# Autodesk Inventor assembly: Robot
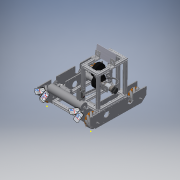
[picture p0: Inventor's stored thumbnail of the model, 180x180]
Saved by Autodesk Inventor 2017 (Build 210142000, 142)
## iProperties
Created: 2016-10-08
Part Number: Robot
Document SubType Name: Assembly
Designer: RoboticsUser
Author: RoboticsUser
## Documents named in this file (12)
- C:\Robotics\CAD\2016-17_CAD\Robot - CAD.iam
- C:\Robotics\CAD\COTSParts\Bosch Extrusion\Gusset 20x20 w screws.ipt
- C:\Robotics\CAD\COTSParts\Bosch Extrusion\Bosch 20x20 9 in - Copy.ipt
- C:\Robotics\CAD\COTSParts\Bosch Extrusion\Rexroth-6mmT-Nutm4.ipt
- C:\Robotics\CAD\COTSParts\Bosch Extrusion\Bosch 20x20 8.937in.ipt
- C:\Robotics\CAD\2016-17_CAD\ParticleLauncher2.0.iam
- C:\Robotics\CAD\2016-17_CAD\Deflecter.ipt
- C:\Robotics\CAD\COTSParts\Actobotics\585 parts\585424.ipt
- C:\Robotics\CAD\2016-17_CAD\WheelAssemble2.0.iam
- C:\Robotics\CAD\2016-17_CAD\RollerHolder.ipt
- C:\Robotics\CAD\2016-17_CAD\NewRoller.ipt
- C:\Robotics\CAD\COTSParts\Bosch Extrusion\Bosch 20x20 9 real.ipt
## Components (21 placed, 11 different names)
1. Bosch 20x20 9 in - Copy:1 — Mate:33, Flush:25, Flush:150, Mate:248, Flush:151, Flush:152, Mate:251, Flush:156, Flush:157, Mate:252, Flush:158
2. Rexroth-6mmT-Nutm4:1
3. Rexroth-6mmT-Nutm4:2 — Mate:33, Flush:25
4. Rexroth-6mmT-Nutm4:3
5. Bosch 20x20 9 in - Copy:2 — Mate:15, Flush:11, Mate:249, Flush:153, Flush:154, Mate:250, Flush:155, Flush:159
6. Rexroth-6mmT-Nutm4:4 — Insert:14
7. Rexroth-6mmT-Nutm4:5
8. Rexroth-6mmT-Nutm4:6 — Mate:15, Flush:11
9. Bosch 20x20 8.937in:4 — Mate:93, Flush:62, Flush:92, Flush:103, Flush:104, Mate:160
10. ParticleLauncher2.0:1 [sub-assembly] — Flush:103, Flush:104, Mate:160, Mate:174, Flush:113, Mate:245, Flush:144, Flush:145
11. Gusset 20x20 w screws:18 — Mate:93, Flush:62, Flush:92
12. Deflecter:2 — Mate:174, Mate:177, Flush:112, Mate:179
13. 585424:2 — Flush:112, Mate:179, Flush:113
14. 585424:3 — Mate:177
15. WheelAssemble2.0:1 [sub-assembly] — Insert:14, Mate:245, Flush:144, Flush:145, Mate:247, Flush:148, Flush:149, Flush:154, Mate:250, Flush:155
16. WheelAssemble2.0:2 [sub-assembly] — Mate:246, Flush:146, Flush:147, Flush:150, Mate:252, Flush:158
17. RollerHolder:1 — Mate:246, Flush:146, Flush:147, Insert:15
18. RollerHolder:2 — Mate:247, Flush:148, Flush:149
19. NewRoller:1 — Insert:15
20. Bosch 20x20 9 real:1 — Mate:251, Flush:156, Flush:157
21. Bosch 20x20 9 real:2 — Mate:248, Flush:151, Flush:152, Mate:249, Flush:153, Flush:159
## Relationships (41: Flush 24, Mate 15, Insert 2)
- Mate:15: Bosch 20x20 9 in - Copy:2 ↔ Rexroth-6mmT-Nutm4:6
- Flush:11 (64.77 mm): Bosch 20x20 9 in - Copy:2 ↔ Rexroth-6mmT-Nutm4:6
- Mate:33: Bosch 20x20 9 in - Copy:1 ↔ Rexroth-6mmT-Nutm4:2
- Flush:25 (64.77 mm): Bosch 20x20 9 in - Copy:1 ↔ Rexroth-6mmT-Nutm4:2
- Mate:93: Bosch 20x20 8.937in:4 ↔ Gusset 20x20 w screws:18
- Flush:62: Bosch 20x20 8.937in:4 ↔ Gusset 20x20 w screws:18
- Flush:92: Bosch 20x20 8.937in:4 ↔ Gusset 20x20 w screws:18
- Flush:103: Bosch 20x20 8.937in:4 ↔ ParticleLauncher2.0:1
- Flush:104: Bosch 20x20 8.937in:4 ↔ ParticleLauncher2.0:1
- Mate:160: Bosch 20x20 8.937in:4 ↔ ParticleLauncher2.0:1
- Mate:174: ParticleLauncher2.0:1 ↔ Deflecter:2
- Mate:177: Deflecter:2 ↔ 585424:3
- Flush:112 (2.54 mm): Deflecter:2 ↔ 585424:2
- Mate:179: Deflecter:2 ↔ 585424:2
- Flush:113 (-88.9 mm): ParticleLauncher2.0:1 ↔ 585424:2
- Insert:14: Rexroth-6mmT-Nutm4:4 ↔ WheelAssemble2.0:1
- Mate:245: ParticleLauncher2.0:1 ↔ WheelAssemble2.0:1
- Flush:144: ParticleLauncher2.0:1 ↔ WheelAssemble2.0:1
- Flush:145 (57.15 mm): ParticleLauncher2.0:1 ↔ WheelAssemble2.0:1
- Mate:246: WheelAssemble2.0:2 ↔ RollerHolder:1
- Flush:146 (18.796 mm): WheelAssemble2.0:2 ↔ RollerHolder:1
- Flush:147: WheelAssemble2.0:2 ↔ RollerHolder:1
- Mate:247: WheelAssemble2.0:1 ↔ RollerHolder:2
- Flush:148: WheelAssemble2.0:1 ↔ RollerHolder:2
- Flush:149 (18.796 mm): WheelAssemble2.0:1 ↔ RollerHolder:2
- Insert:15: RollerHolder:1 ↔ NewRoller:1
- Flush:150: Bosch 20x20 9 in - Copy:1 ↔ WheelAssemble2.0:2
- Mate:248: Bosch 20x20 9 in - Copy:1 ↔ Bosch 20x20 9 real:2
- Flush:151: Bosch 20x20 9 in - Copy:1 ↔ Bosch 20x20 9 real:2
- Flush:152: Bosch 20x20 9 in - Copy:1 ↔ Bosch 20x20 9 real:2
- Mate:249: Bosch 20x20 9 in - Copy:2 ↔ Bosch 20x20 9 real:2
- Flush:153: Bosch 20x20 9 in - Copy:2 ↔ Bosch 20x20 9 real:2
- Flush:154: Bosch 20x20 9 in - Copy:2 ↔ WheelAssemble2.0:1
- Mate:250: Bosch 20x20 9 in - Copy:2 ↔ WheelAssemble2.0:1
- Flush:155 (-38.1 mm): Bosch 20x20 9 in - Copy:2 ↔ WheelAssemble2.0:1
- Mate:251: Bosch 20x20 9 in - Copy:1 ↔ Bosch 20x20 9 real:1
- Flush:156: Bosch 20x20 9 in - Copy:1 ↔ Bosch 20x20 9 real:1
- Flush:157: Bosch 20x20 9 in - Copy:1 ↔ Bosch 20x20 9 real:1
- Mate:252: Bosch 20x20 9 in - Copy:1 ↔ WheelAssemble2.0:2
- Flush:158 (38.1 mm): Bosch 20x20 9 in - Copy:1 ↔ WheelAssemble2.0:2
- Flush:159: Bosch 20x20 9 in - Copy:2 ↔ Bosch 20x20 9 real:2
